# Autodesk Inventor assembly: 20X20lift
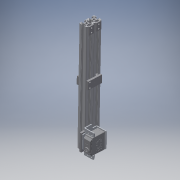
[picture p0: Inventor's stored thumbnail of the model, 180x180]
Saved by Autodesk Inventor 2017 SP1 (Build 210196100, 196)
## iProperties
Created: 2017-12-15
Part Number: 20X20lift
Document SubType Name: Assembly
Designer: User
Author: User
## Documents named in this file (7)
- C:\robotics\CAD\2017-18_CAD\20X20lift.iam
- C:\robotics\CAD\2017-18_CAD\Prototypes\Sliderfor2020.ipt
- C:\robotics\CAD\COTSParts\Bosch Extrusion\Bosch 20x20 11.ipt
- C:\robotics\CAD\2017-18_CAD\Prototypes\ServosSlideforLift.ipt
- C:\robotics\CAD\COTSParts\Tetrix\39060_txm-standard servo bracket.ipt
- C:\robotics\CAD\2017-18_CAD\ShoulderScrewHolderSlide.ipt
- C:\robotics\CAD\COTSParts\Rev\REV-41-1097.ipt
## Components (9 placed, 6 different names)
1. Sliderfor2020:2 — Mate:10, Mate:11
2. Sliderfor2020:3 — Mate:5, Mate:6, Mate:8, Mate:9
3. Bosch 20x20 11:1 — Mate:5, Mate:6, Mate:11, Mate:16, Flush:3, Flush:4, Flush:5
4. Bosch 20x20 11:2 — Mate:8, Mate:9, Mate:10, Mate:15, Flush:1, Flush:2, Flush:5, Flush:6, Mate:21, Mate:22
5. ServosSlideforLift:1 — Mate:21, Mate:22, Insert:3, Angle:1
6. 39060_txm-standard servo bracket:1 — Flush:6, Insert:1, Insert:2, Insert:3, Angle:1
7. ShoulderScrewHolderSlide:1 — Mate:15, Flush:1, Flush:2
8. ShoulderScrewHolderSlide:2 — Mate:16, Flush:3, Flush:4
9. REV-41-1097:1 — Insert:1, Insert:2
## Relationships (20: Mate 10, Flush 6, Insert 3, Angle 1)
- Mate:5: Sliderfor2020:3 ↔ Bosch 20x20 11:1
- Mate:6: Sliderfor2020:3 ↔ Bosch 20x20 11:1
- Mate:8: Sliderfor2020:3 ↔ Bosch 20x20 11:2
- Mate:9: Sliderfor2020:3 ↔ Bosch 20x20 11:2
- Mate:10: Sliderfor2020:2 ↔ Bosch 20x20 11:2
- Mate:11: Sliderfor2020:2 ↔ Bosch 20x20 11:1
- Mate:15: Bosch 20x20 11:2 ↔ ShoulderScrewHolderSlide:1
- Flush:1: Bosch 20x20 11:2 ↔ ShoulderScrewHolderSlide:1
- Flush:2 (3.81 mm): Bosch 20x20 11:2 ↔ ShoulderScrewHolderSlide:1
- Mate:16: Bosch 20x20 11:1 ↔ ShoulderScrewHolderSlide:2
- Flush:3: Bosch 20x20 11:1 ↔ ShoulderScrewHolderSlide:2
- Flush:4 (3.81 mm): Bosch 20x20 11:1 ↔ ShoulderScrewHolderSlide:2
- Flush:5: Bosch 20x20 11:1 ↔ Bosch 20x20 11:2
- Flush:6: Bosch 20x20 11:2 ↔ 39060_txm-standard servo bracket:1
- Mate:21: Bosch 20x20 11:2 ↔ ServosSlideforLift:1
- Mate:22: Bosch 20x20 11:2 ↔ ServosSlideforLift:1
- Insert:1: 39060_txm-standard servo bracket:1 ↔ REV-41-1097:1
- Insert:2: 39060_txm-standard servo bracket:1 ↔ REV-41-1097:1
- Insert:3: ServosSlideforLift:1 ↔ 39060_txm-standard servo bracket:1
- Angle:1 (0 deg): ServosSlideforLift:1 ↔ 39060_txm-standard servo bracket:1
